# Autodesk Inventor assembly: Lift - Routing Sprocket
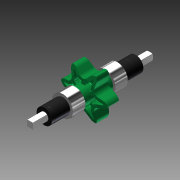
[picture p0: Inventor's stored thumbnail of the model, 180x180]
Saved by Autodesk Inventor 2012 (Build 160160000, 160)
## iProperties
Created: 2011-09-11
Part Number: Lift - Routing Sprocket
Document SubType Name: Assembly
Designer: Wade
Author: Wade
## Documents named in this file (6)
- C:\Users\Wade\Documents\1103 Robot - CAD Assembly\Lift - Routing Sprocket.iam
- C:\Users\Wade\Documents\24C VEX CAD Files\Drive Shafts\Drive Shaft (Square Bar) 2.5''.ipt
- C:\Users\Wade\Documents\24C VEX CAD Files\Gears & Pulleys\High Strength 6-Tooth Sprocket.ipt
- C:\Users\Wade\Documents\24C VEX CAD Files\Other Parts\Shaft Collar (with Set Screw Installed).ipt
- C:\Users\Wade\Documents\24C VEX CAD Files\Washers & Spacers\Spacer (Thin), 4.6mm.ipt
- C:\Users\Wade\Documents\24C VEX CAD Files\Washers & Spacers\Spacer (Thick), 8mm.ipt
## Components (8 placed, 5 different names)
1. Drive Shaft (Square Bar) 2.5'':1 — Mate:1, Mate:2, Flush:1, Flush:2, Flush:4, Flush:5
2. High Strength 6-Tooth Sprocket:1 — Mate:1, Mate:2, Flush:1, Mate:3, Mate:4, Mate:5, Mate:6, Mate:8, Mate:11
3. Shaft Collar (with Set Screw Installed):1 — Flush:2, Mate:3, Mate:4, Flush:3, Mate:10
4. Shaft Collar (with Set Screw Installed):2 — Mate:5, Mate:6, Flush:3, Mate:7
5. Spacer (Thin), 4.6mm:1 — Mate:9, Flush:4
6. Spacer (Thick), 8mm:1 — Mate:7, Mate:8, Mate:9
7. Spacer (Thick), 8mm:2 — Mate:10, Mate:11, Mate:12
8. Spacer (Thin), 4.6mm:2 — Mate:12, Flush:5
## Relationships (17: Mate 12, Flush 5)
- Mate:1: Drive Shaft (Square Bar) 2.5'':1 ↔ High Strength 6-Tooth Sprocket:1
- Mate:2: Drive Shaft (Square Bar) 2.5'':1 ↔ High Strength 6-Tooth Sprocket:1
- Flush:1 (23.8125 mm): Drive Shaft (Square Bar) 2.5'':1 ↔ High Strength 6-Tooth Sprocket:1
- Flush:2: Drive Shaft (Square Bar) 2.5'':1 ↔ Shaft Collar (with Set Screw Installed):1
- Mate:3: High Strength 6-Tooth Sprocket:1 ↔ Shaft Collar (with Set Screw Installed):1
- Mate:4: High Strength 6-Tooth Sprocket:1 ↔ Shaft Collar (with Set Screw Installed):1
- Mate:5: High Strength 6-Tooth Sprocket:1 ↔ Shaft Collar (with Set Screw Installed):2
- Mate:6: High Strength 6-Tooth Sprocket:1 ↔ Shaft Collar (with Set Screw Installed):2
- Flush:3: Shaft Collar (with Set Screw Installed):1 ↔ Shaft Collar (with Set Screw Installed):2
- Mate:7: Shaft Collar (with Set Screw Installed):2 ↔ Spacer (Thick), 8mm:1
- Mate:8: High Strength 6-Tooth Sprocket:1 ↔ Spacer (Thick), 8mm:1
- Mate:9: Spacer (Thin), 4.6mm:1 ↔ Spacer (Thick), 8mm:1
- Flush:4 (7.5184 mm): Drive Shaft (Square Bar) 2.5'':1 ↔ Spacer (Thin), 4.6mm:1
- Mate:10: Shaft Collar (with Set Screw Installed):1 ↔ Spacer (Thick), 8mm:2
- Mate:11: High Strength 6-Tooth Sprocket:1 ↔ Spacer (Thick), 8mm:2
- Mate:12: Spacer (Thick), 8mm:2 ↔ Spacer (Thin), 4.6mm:2
- Flush:5 (7.5184 mm): Drive Shaft (Square Bar) 2.5'':1 ↔ Spacer (Thin), 4.6mm:2
